# Autodesk Inventor assembly: Ascensor uvas + riel1
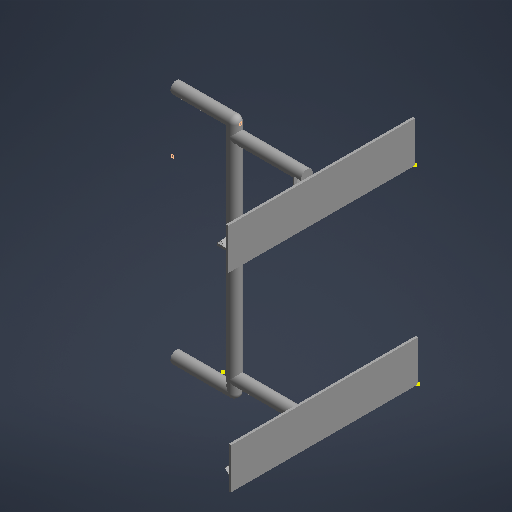
[picture p0: Inventor's stored thumbnail of the model, 512x512]
Saved by Autodesk Inventor 2026.2 (Build 302298010, 298A)
## iProperties
Part Number: Ascensor uvas + riel1
Document SubType Name: Assembly
Designer: diego
Author: diego
## Documents named in this file (7)
- C:\Proyectos\Inventor\Piezas, ensambles y planos\Uvas.v2\Ascensor uvas + riel1.iam
- C:\Proyectos\Inventor\Piezas, ensambles y planos\Uvas.v2\Union_Poleas.ipt
- C:\Proyectos\Inventor\Piezas, ensambles y planos\Uvas.v2\Rueda.ipt
- C:\Proyectos\Inventor\Piezas, ensambles y planos\Uvas.v2\ISO 4014 - M14 x 90 - ISO.ipt
- C:\Proyectos\Inventor\Piezas, ensambles y planos\Uvas.v2\ISO 4161 - M14(1).ipt
- C:\Proyectos\Inventor\Piezas, ensambles y planos\Uvas.v2\Riel superior.ipt
- C:\Proyectos\Inventor\Piezas, ensambles y planos\Uvas.v2\Riel Inferior.ipt
## Components (9 placed, 6 different names)
1. Union_Poleas:1 — Coincidencia:1, Coincidencia:2, Coincidencia:3, Coincidencia:4, De rotación:2, Coincidencia:5, Coincidencia:6, Coincidencia:7, Coincidencia:8, De rotación:3, De rotación:4
2. Rueda:2 — De rotación:2, De rotación:4
3. ISO 4014 M14 x 90:1 — Coincidencia:1, Coincidencia:2
4. ISO 4161 M14:1 — Coincidencia:3, Coincidencia:4
5. ISO 4014 M14 x 90:2 — Coincidencia:5, Coincidencia:6
6. ISO 4161 M14:2 — Coincidencia:7, Coincidencia:8
7. Rueda:3 — De rotación:3
8. Riel superior:1
9. Riel Inferior:1
## Relationships (11: Mate 8, RevoluteJoint 3)
- Coincidencia:1 [Mate]: Union_Poleas:1 ↔ ISO 4014 M14 x 90:1
- Coincidencia:2 [Mate]: Union_Poleas:1 ↔ ISO 4014 M14 x 90:1
- Coincidencia:3 [Mate]: Union_Poleas:1 ↔ ISO 4161 M14:1
- Coincidencia:4 [Mate]: Union_Poleas:1 ↔ ISO 4161 M14:1
- De rotación:2 [RevoluteJoint]: Union_Poleas:1 ↔ Rueda:2
- Coincidencia:5 [Mate]: Union_Poleas:1 ↔ ISO 4014 M14 x 90:2
- Coincidencia:6 [Mate]: Union_Poleas:1 ↔ ISO 4014 M14 x 90:2
- Coincidencia:7 [Mate]: Union_Poleas:1 ↔ ISO 4161 M14:2
- Coincidencia:8 [Mate]: Union_Poleas:1 ↔ ISO 4161 M14:2
- De rotación:3 [RevoluteJoint]: Union_Poleas:1 ↔ Rueda:3
- De rotación:4 [RevoluteJoint]: Union_Poleas:1 ↔ Rueda:2
